# Autodesk Inventor assembly: Intake new robot
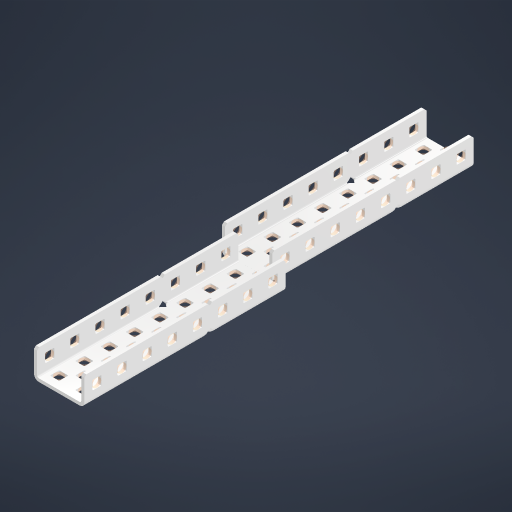
[picture p0: Inventor's stored thumbnail of the model, 512x512]
Saved by Autodesk Inventor 2023 (Build 270158000, 158)
## iProperties
Created: 2023-11-30
Part Number: Intake new robot
Document SubType Name: Assembly
Designer: diego
Author: diego
## Documents named in this file (2)
- C:\Users\diego\OneDrive\Documents\GitHub\2024-599Z\2024-599Z\Cad\Intake new robot.iam
- C:\Users\diego\OneDrive\Documents\GitHub\2024-599Z\2024-599Z\Cad\VEX-CAD-Inventor-1.4.0\Structure\C Channel\Aluminum 1x2x1\Alu C 1x2x1x8.ipt
## Components (2 placed, 1 different names)
1. Alu C 1x2x1x8:1 — Mate:1
2. Alu C 1x2x1x8:2 — Mate:1
## Relationships (1: Mate 1)
- Mate:1: Alu C 1x2x1x8:1 ↔ Alu C 1x2x1x8:2
